# Autodesk Inventor assembly: tandwiel_MIR
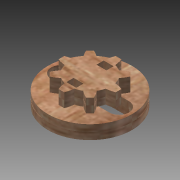
[picture p0: Inventor's stored thumbnail of the model, 180x180]
Saved by Autodesk Inventor 2015 (Build 190159000, 159)
## iProperties
Created: 2016-01-31
Part Number: tandwiel_MIR
Document SubType Name: Assembly
Designer: david
Author: david
## Documents named in this file (3)
- Z:\gip\Inventor\generatie 7\motor\tandwiel\tandwiel_MIR.iam
- Z:\gip\Inventor\generatie 7\motor\tandwiel\1_MIR.ipt
- Z:\gip\Inventor\generatie 7\motor\tandwiel\tandwiel(ja)_MIR.ipt
## Components (4 placed, 2 different names)
1. 1_MIR:1 — Flush:1, Mate:2, Mate:1
2. 1_MIR:2 — Flush:1, Mate:2, Mate:1, Flush:4, Flush:3, Flush:2
3. tandwiel(ja)_MIR:1 — Flush:4, Flush:3, Flush:2, Flush:5, Mate:4, Mate:3
4. tandwiel(ja)_MIR:2 — Flush:5, Mate:4, Mate:3
## Relationships (9: Mate 5, Flush 4)
- Flush:1: 1_MIR:1 ↔ 1_MIR:2
- Mate:2: 1_MIR:1 ↔ 1_MIR:2
- Mate:1: 1_MIR:1 ↔ 1_MIR:2
- Flush:4: 1_MIR:2 ↔ tandwiel(ja)_MIR:1
- Flush:3: 1_MIR:2 ↔ tandwiel(ja)_MIR:1
- Flush:2 [Mate]: 1_MIR:2 ↔ tandwiel(ja)_MIR:1
- Flush:5: tandwiel(ja)_MIR:1 ↔ tandwiel(ja)_MIR:2
- Mate:4: tandwiel(ja)_MIR:1 ↔ tandwiel(ja)_MIR:2
- Mate:3: tandwiel(ja)_MIR:1 ↔ tandwiel(ja)_MIR:2
